# Autodesk Inventor assembly: A2017_T5_03
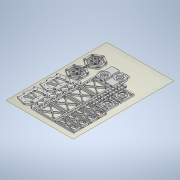
[picture p0: Inventor's stored thumbnail of the model, 180x180]
Saved by Autodesk Inventor 2020 (Build 240168000, 168)
## iProperties
Created: 2021-08-27
Part Number: A2017_T5_03
Document SubType Name: Assembly
Designer: Masato
Author: Masato
## Documents named in this file (11)
- C:\Users\naoki\Documents\Inventor\CitBrains\git_clone\SUSTAINA_ver1_0\AT5_173\SUSTAINA-OP\Cam\A2017_T5_03.iam
- C:\Users\naoki\Documents\Inventor\CitBrains\git_clone\SUSTAINA_ver1_0\AT5_173\SUSTAINA-OP\Cam\DisposableBoard.ipt
- C:\Users\naoki\Documents\Inventor\CitBrains\git_clone\SUSTAINA_ver1_0\AT5_173\SUSTAINA-OP\LowerBody\Knee\Knee_clamp.ipt
- C:\Users\naoki\Documents\Inventor\CitBrains\git_clone\SUSTAINA_ver1_0\AT5_173\SUSTAINA-OP\LowerBody\Foot\Foot_root_block.ipt
- C:\Users\naoki\Documents\Inventor\CitBrains\git_clone\SUSTAINA_ver1_0\AT5_173\SUSTAINA-OP\UpperBody\Trunk\Trunk_lower_side_frame.ipt
- C:\Users\naoki\Documents\Inventor\CitBrains\git_clone\SUSTAINA_ver1_0\AT5_173\SUSTAINA-OP\UpperBody\Arm\Shoulder_horn_frame.ipt
- C:\Users\naoki\Documents\Inventor\CitBrains\git_clone\SUSTAINA_ver1_0\AT5_173\SUSTAINA-OP\LowerBody\Link\FrontLink_diagonal.ipt
- C:\Users\naoki\Documents\Inventor\CitBrains\git_clone\SUSTAINA_ver1_0\AT5_173\SUSTAINA-OP\LowerBody\Link\BackLink_diagonal.ipt
- C:\Users\naoki\Documents\Inventor\CitBrains\git_clone\SUSTAINA_ver1_0\AT5_173\SUSTAINA-OP\UpperBody\Trunk\CrossRollerBearing\Outer_support_stand.ipt
- C:\Users\naoki\Documents\Inventor\CitBrains\git_clone\SUSTAINA_ver1_0\AT5_173\SUSTAINA-OP\UpperBody\Trunk\CrossRollerBearing\Inner_support_stand.ipt
- C:\Users\naoki\Documents\Inventor\CitBrains\git_clone\SUSTAINA_ver1_0\AT5_173\SUSTAINA-OP\LowerBody\Leg_joint\Leg_joint_yaw_frame.ipt
## Components (35 placed, 10 different names)
1. DisposableBoard:1 — メイト:2, メイト:1, フラッシュ:1, フラッシュ:2, メイト:4, メイト:5, メイト:6, メイト:7, メイト:9, フラッシュ:4, フラッシュ:7, 正接:1, 角度:1, フラッシュ:8, メイト:13, 正接:3, メイト:20, メイト:21, メイト:24, メイト:25, 角度:2, 角度:4, 正接:6
2. Leg_joint_yaw_frame:1 — メイト:25, メイト:26, 正接:8, フラッシュ:9
3. Leg_joint_yaw_frame:2 — メイト:24, メイト:27, 正接:8
4. FrontLink_diagonal:1 — メイト:6, フラッシュ:4, 正接:4, メイト:18
5. FrontLink_diagonal:2
6. FrontLink_diagonal:3 — メイト:19
7. FrontLink_diagonal:4 — メイト:26, メイト:27, フラッシュ:9
8. BackLink_diagonal:1 — メイト:5, フラッシュ:7, メイト:18
9. BackLink_diagonal:2
10. BackLink_diagonal:3
11. BackLink_diagonal:4 — メイト:14, メイト:16
12. Trunk_lower_side_frame:1 — メイト:4, 正接:1, フラッシュ:8, 正接:2
13. Trunk_lower_side_frame:2 — 正接:5
14. Foot_root_block:1 — メイト:9, メイト:16, メイト:19
15. Foot_root_block:2
16. Foot_root_block:3
17. Foot_root_block:4
18. Foot_root_block:5
19. Foot_root_block:6
20. Foot_root_block:7 — メイト:17
21. Foot_root_block:8
22. Knee_clamp:1 — メイト:7, 角度:1, 正接:2, 正接:3, 正接:4
23. Knee_clamp:2
24. Knee_clamp:3
25. Knee_clamp:4
26. Knee_clamp:5
27. Knee_clamp:6
28. Knee_clamp:7
29. Knee_clamp:8
30. Shoulder_horn_frame:2 — メイト:13, メイト:14, メイト:17
31. Shoulder_horn_frame:3
32. Inner_support_stand:1 — メイト:20, 角度:4, 正接:7
33. Outer_support_stand:1 — メイト:21, 角度:2, 正接:5, 正接:6, 正接:7
34. Inner_support_stand:2
35. Outer_support_stand:2
## Component patterns: (4 elements, first: FrontLink_diagonal:1), (4 elements, first: BackLink_diagonal:1), (2 elements, first: Trunk_lower_side_frame:1), (8 elements, first: Foot_root_block:1), (8 elements, first: Knee_clamp:1), (2 elements, first: Shoulder_horn_frame:2), (2 elements, first: Inner_support_stand:1 + Outer_support_stand:1)
## Relationships (36: Mate 19, Tangent 8, Flush 6, Angle 3)
- メイト:2 [Mate]: DisposableBoard:1
- メイト:1 [Mate]: DisposableBoard:1
- フラッシュ:1 [Flush]: DisposableBoard:1
- フラッシュ:2 [Flush]: DisposableBoard:1
- メイト:4 [Mate]: DisposableBoard:1 ↔ Trunk_lower_side_frame:1
- メイト:5 [Mate]: DisposableBoard:1 ↔ BackLink_diagonal:1
- メイト:6 [Mate]: DisposableBoard:1 ↔ FrontLink_diagonal:1
- メイト:7 [Mate]: DisposableBoard:1 ↔ Knee_clamp:1
- メイト:9 [Mate]: DisposableBoard:1 ↔ Foot_root_block:1
- フラッシュ:4 [Flush] (2 mm): DisposableBoard:1 ↔ FrontLink_diagonal:1
- フラッシュ:7 [Flush] (2 mm): DisposableBoard:1 ↔ BackLink_diagonal:1
- 正接:1 [Tangent] (2 mm): DisposableBoard:1 ↔ Trunk_lower_side_frame:1
- 角度:1 [Angle] (45 deg): DisposableBoard:1 ↔ Knee_clamp:1
- フラッシュ:8 [Flush] (2 mm): DisposableBoard:1 ↔ Trunk_lower_side_frame:1
- メイト:13 [Mate]: DisposableBoard:1 ↔ Shoulder_horn_frame:2
- メイト:14 [Mate] (2.5 mm): BackLink_diagonal:4 ↔ Shoulder_horn_frame:2
- メイト:16 [Mate] (2.5 mm): BackLink_diagonal:4 ↔ Foot_root_block:1
- メイト:17 [Mate] (2.5 mm): Foot_root_block:7 ↔ Shoulder_horn_frame:2
- 正接:2 [Tangent] (2.5 mm): Trunk_lower_side_frame:1 ↔ Knee_clamp:1
- 正接:3 [Tangent] (2 mm): DisposableBoard:1 ↔ Knee_clamp:1
- 正接:4 [Tangent] (2.5 mm): FrontLink_diagonal:1 ↔ Knee_clamp:1
- メイト:18 [Mate] (2.5 mm): FrontLink_diagonal:1 ↔ BackLink_diagonal:1
- メイト:19 [Mate] (2.5 mm): FrontLink_diagonal:3 ↔ Foot_root_block:1
- メイト:20 [Mate]: DisposableBoard:1 ↔ Inner_support_stand:1
- メイト:21 [Mate]: DisposableBoard:1 ↔ Outer_support_stand:1
- メイト:24 [Mate]: DisposableBoard:1 ↔ Leg_joint_yaw_frame:2
- メイト:25 [Mate]: DisposableBoard:1 ↔ Leg_joint_yaw_frame:1
- 角度:2 [Angle] (0 deg): DisposableBoard:1 ↔ Outer_support_stand:1
- 角度:4 [Angle] (0 deg): DisposableBoard:1 ↔ Inner_support_stand:1
- 正接:5 [Tangent] (2.5 mm): Trunk_lower_side_frame:2 ↔ Outer_support_stand:1
- 正接:6 [Tangent] (4 mm): DisposableBoard:1 ↔ Outer_support_stand:1
- 正接:7 [Tangent] (-4 mm): Inner_support_stand:1 ↔ Outer_support_stand:1
- メイト:26 [Mate] (2.5 mm): Leg_joint_yaw_frame:1 ↔ FrontLink_diagonal:4
- メイト:27 [Mate] (2.5 mm): Leg_joint_yaw_frame:2 ↔ FrontLink_diagonal:4
- 正接:8 [Tangent] (2.5 mm): Leg_joint_yaw_frame:1 ↔ Leg_joint_yaw_frame:2
- フラッシュ:9 [Flush]: Leg_joint_yaw_frame:1 ↔ FrontLink_diagonal:4
